# Autodesk Inventor assembly: LeftUpperLimbBlock
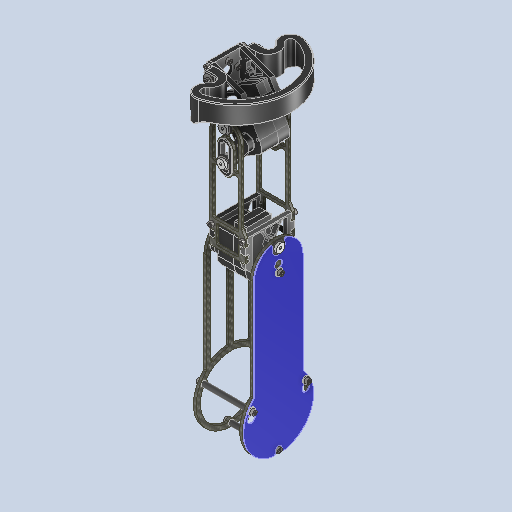
[picture p0: Inventor's stored thumbnail of the model, 512x512]
Saved by Autodesk Inventor 2024.2 (Build 282272000, 272)
## iProperties
Created: 2024-01-18
Part Number: LeftUpperLimbBlock
Document SubType Name: Assembly
Designer: Masato Kubotera
Mass: 424.438 g
Surface Area: 1330.22 cm^2
Volume: 215.834 cm^3
Author: Masato Kubotera
## Documents named in this file (6)
- C:\Users\masato\OneDrive - Chiba Institute of Technology\CIT Brains\RoboCup2024\Mechanic\SUSTAINA-OP2-DEV1\NativeFiles\Boby\UpperLimb\LeftUpperLimbBlock.iam
- C:\Users\masato\OneDrive - Chiba Institute of Technology\CIT Brains\RoboCup2024\Mechanic\SUSTAINA-OP2-DEV1\NativeFiles\Boby\UpperLimb\Shoulders\LeftShoulderUnit.iam
- C:\Users\masato\OneDrive - Chiba Institute of Technology\CIT Brains\RoboCup2024\Mechanic\SUSTAINA-OP2-DEV1\NativeFiles\Boby\UpperLimb\UpperArms\LeftUpperArmUnit.iam
- C:\Users\masato\OneDrive - Chiba Institute of Technology\CIT Brains\RoboCup2024\Mechanic\SUSTAINA-OP2-DEV1\NativeFiles\Boby\UpperLimb\LowerArms\LeftLowerArmUnit.iam
- C:\Users\masato\OneDrive - Chiba Institute of Technology\CIT Brains\RoboCup2024\Mechanic\SUSTAINA-OP2-DEV1\NativeFiles\Boby\UpperLimb\UpperArms\LeftUpperArmCrankUnit.iam
- C:\Users\masato\OneDrive - Chiba Institute of Technology\CIT Brains\RoboCup2024\Mechanic\SUSTAINA-OP2-DEV1\NativeFiles\Boby\UpperLimb\Shoulders\LeftShoulderCrankUnit.iam
## Components (5 placed, 5 different names)
1. LeftShoulderUnit:1 [sub-assembly] — Shoulder-Pitch, Shoulder-Roll, [Auto]Shoulder-Roll-Crank, Mate:1, Mate:2, Insert:1, Insert:2, Insert:3
2. LeftShoulderCrankUnit:1 [sub-assembly] — Insert:1, [Auto]Shoulder-Roll-Crank
3. LeftUpperArmUnit:1 [sub-assembly] — Insert:2, Insert:3, Shoulder-Roll, Insert:4, Insert:5, Insert:6, Elbow-Pitch, [Auto]Elbow-Pitch
4. LeftUpperArmCrankUnit:1 [sub-assembly] — Insert:5, [Auto]Elbow-Pitch
5. LeftLowerArmUnit:1 [sub-assembly] — Insert:4, Insert:6, Elbow-Pitch
## Relationships (13: Insert 6, Angle 5, Mate 2)
- Shoulder-Pitch [Angle] (0 deg): LeftShoulderUnit:1
- Shoulder-Roll [Angle] (0 deg): LeftShoulderUnit:1 ↔ LeftUpperArmUnit:1
- Elbow-Pitch [Angle] (0 deg): LeftUpperArmUnit:1 ↔ LeftLowerArmUnit:1
- [Auto]Shoulder-Roll-Crank [Angle] (-180 deg): LeftShoulderUnit:1 ↔ LeftShoulderCrankUnit:1
- [Auto]Elbow-Pitch [Angle] (-180 deg): LeftUpperArmUnit:1 ↔ LeftUpperArmCrankUnit:1
- Mate:1: LeftShoulderUnit:1
- Mate:2: LeftShoulderUnit:1
- Insert:1: LeftShoulderUnit:1 ↔ LeftShoulderCrankUnit:1
- Insert:2: LeftShoulderUnit:1 ↔ LeftUpperArmUnit:1
- Insert:3: LeftShoulderUnit:1 ↔ LeftUpperArmUnit:1
- Insert:4: LeftUpperArmUnit:1 ↔ LeftLowerArmUnit:1
- Insert:5: LeftUpperArmUnit:1 ↔ LeftUpperArmCrankUnit:1
- Insert:6: LeftUpperArmUnit:1 ↔ LeftLowerArmUnit:1
